# Autodesk Inventor assembly: Bottom Assembly
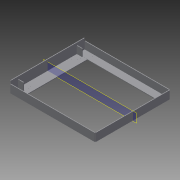
[picture p0: Inventor's stored thumbnail of the model, 180x180]
Saved by Autodesk Inventor 2015 (Build 190159000, 159)
## iProperties
Created: 2017-01-05
Part Number: Bottom Assembly
Document SubType Name: Weldment
Designer: ps2du
Weld Material: Welded Aluminum-6061
Author: ps2du
## Documents named in this file (6)
- E:\Robo Parts Inventor\Bottom Assembly.iam
- E:\Robo Parts Inventor\14in L Channel.ipt
- E:\Robo Parts Inventor\16in L Channel.ipt
- E:\Robo Parts Inventor\14in 2inL Channel.ipt
- E:\Robo Parts Inventor\14in L Mount.ipt
- E:\Robo Parts Inventor\14in L Mount_MIR.ipt
## Components (6 placed, 5 different names)
1. 14in L Channel:1 — Rigid:2, Rigid:3
2. 16in L Channel:1 — Rigid:2, Symmetry:1
3. 16in L Channel:2 — Rigid:3, Rigid:4, Symmetry:1
4. 14in 2inL Channel:1 — Rigid:4, Rigid:5
5. 14in L Mount:2 — Rigid:5
6. 14in L Mount_MIR:1
## Relationships (5: WeldJoint 4, Symmetry 1)
- Rigid:2 [WeldJoint]: 14in L Channel:1 ↔ 16in L Channel:1
- Rigid:3 [WeldJoint]: 14in L Channel:1 ↔ 16in L Channel:2
- Rigid:4 [WeldJoint]: 16in L Channel:2 ↔ 14in 2inL Channel:1
- Rigid:5 [WeldJoint] (-38.1 mm): 14in 2inL Channel:1 ↔ 14in L Mount:2
- Symmetry:1: 16in L Channel:1 ↔ 16in L Channel:2
